# Autodesk Inventor assembly: Редуктор
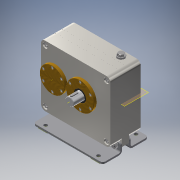
[picture p0: Inventor's stored thumbnail of the model, 180x180]
Saved by Autodesk Inventor 2016 (Build 200138000, 138)
## iProperties
Created: 2021-04-28
Part Number: Редуктор
Material: Типовые
Document SubType Name: Assembly
Designer: Лол
Mass: 4191.1 g
Surface Area: 9151.06 cm^2
Volume: 3369.82 cm^3
Density: 1.24372 g/cm^3
Author: Лол
## Documents named in this file (36)
- C:\Users\Лол\Documents\Inventor\course_work\Редуктор.iam
- C:\Users\Лол\Documents\Inventor\course_work\Корпус часть без резьбы.ipt
- C:\Users\Лол\Documents\Inventor\course_work\Подшипник\Подшипник-01.ipt
- C:\Users\Лол\Documents\Inventor\course_work\Подшипник.ipt
- C:\Users\Лол\Documents\Inventor\course_work\Подшипник\Подшипник-02.ipt
- C:\Users\Лол\Documents\Inventor\course_work\Быстроходный вал.ipt
- C:\Users\Лол\Documents\Inventor\course_work\Тихоходный вал.ipt
- C:\Users\Лол\Documents\Inventor\course_work\Кольцо A30 ГОСТ 13942-86.ipt
- C:\Users\Лол\Documents\Inventor\course_work\Кольцо A35 ГОСТ 13942-86.ipt
- C:\Users\Лол\Documents\Inventor\course_work\Тихоходное колесо.ipt
- C:\Users\Лол\Documents\Inventor\course_work\Корпус центральная часть.ipt
- C:\Users\Лол\Documents\Inventor\course_work\Корпус часть с резьбой.ipt
- C:\Users\Лол\Documents\Inventor\course_work\Гайка M30x1.5 6H ГОСТ 6393-73.ipt
- C:\Users\Лол\Documents\Inventor\course_work\Гайка M33x1.5 6H ГОСТ 6393-73.ipt
- C:\Users\Лол\Documents\Inventor\course_work\ISO 2340 - A - 6 x 40ISO.ipt
- C:\Users\Лол\Documents\Inventor\course_work\AS 1420 - 1973 - M10 x 75.ipt
- C:\Users\Лол\Documents\Inventor\course_work\Крышка маленькая_62.ipt
- C:\Users\Лол\Documents\Inventor\course_work\Крышка большая_72.ipt
- C:\Users\Лол\Documents\Inventor\course_work\AS 1420 - 1973 - M6 x 12.ipt
- C:\Users\Лол\Documents\Inventor\course_work\Крышка маленькая_под манж_01.ipt
- C:\Users\Лол\Documents\Inventor\course_work\Крышка большая_ПОД МАНЖЕТУ.ipt
- C:\Users\Лол\Documents\Inventor\course_work\Манжет 1-28x40x7 ГОСТ 8752-79.ipt
- C:\Users\Лол\Documents\Inventor\course_work\Манжет 1-30x42x7 ГОСТ 8752-79.ipt
- C:\Users\Лол\Documents\Inventor\course_work\ОПОРА_05.ipt
- C:\Users\Лол\Documents\Inventor\course_work\Шпонка 8x7x28 ГОСТ 23360-78.ipt
- C:\Users\Лол\Documents\Inventor\course_work\Болт 2 M10×50 ГОСТ 15591-70.ipt
- C:\Users\Лол\Documents\Inventor\course_work\Гайка M10-6H ГОСТ 5927-70.ipt
- C:\Users\Лол\Documents\Inventor\course_work\Шайба 2 10Л ГОСТ 6402-78.ipt
- C:\Users\Лол\Documents\Inventor\course_work\кол_062.ipt
- C:\Users\Лол\Documents\Inventor\course_work\кол_072.ipt
- C:\Users\Лол\Documents\Inventor\course_work\CSN 02 1915.21 - M 20 x 10.ipt
- C:\Users\Лол\Documents\Inventor\course_work\DIN 7603 - A22 x 27  (lt).ipt
- C:\Users\Лол\Documents\Inventor\course_work\платик под опору редуктора-01.ipt
- C:\Users\Лол\Documents\Inventor\course_work\Кольцо C6 ГОСТ 13942-86.ipt
- C:\Users\Лол\Documents\Inventor\course_work\ISO 2340 - A - 6 x 45ISO.ipt
- C:\Users\Лол\Documents\Inventor\course_work\сапун - M 20 x 10.ipt
## Components (82 placed, 33 different names)
1. Корпус часть без резьбы:1 — Заподлицо:1, Заподлицо:2, Заподлицо:3, Совмещение:1, Совмещение:2, Совмещение:3, Совмещение:4, Совмещение:14, Совмещение:28, Совмещение:33, Совмещение:34, Совмещение:35, Совмещение:36, Совмещение:37, Совмещение:38, Совмещение:39, Совмещение:40, Совмещение:43, Совмещение:44, Совмещение:61, Совмещение:62, Совмещение:82, Совмещение:83, Совмещение:84, Совмещение:191, Заподлицо:10, Совмещение:192, Заподлицо:11, Угол:1, Совмещение:215, Угол:14, Угол:15, Угол:16, Угол:17, Угол:18, Угол:19, Угол:20, Угол:21, Угол:22, Угол:23, Угол:27
2. Подшипник-01:1 — Совмещение:18, Совмещение:19, Совмещение:22, Совмещение:24, Совмещение:221
3. Подшипник-01:2 — Совмещение:1, Совмещение:2, Совмещение:5, Совмещение:13, Совмещение:222
4. Подшипник-02:3 — Совмещение:3, Совмещение:4, Совмещение:6, Совмещение:26, Совмещение:223
5. Подшипник-02:4 — Совмещение:16, Совмещение:17, Совмещение:, Совмещение:88, Совмещение:220
6. Быстроходный вал:1 — Совмещение:5, Совмещение:7, Совмещение:8, Совмещение:22, Совмещение:23, Совмещение:85, Совмещение:109, Совмещение:159, Совмещение:160, Угол:29
7. Тихоходный вал:1 — Совмещение:6, Совмещение:9, Совмещение:12, Совмещение:25, Совмещение:48, Совмещение:87, Совмещение:88, Совмещение:112, Совмещение:157, Совмещение:158
8. Кольцо A30 ГОСТ 13942-86:1 — Совмещение:7, Совмещение:8, Совмещение:13, Угол:27
9. Кольцо A35 ГОСТ 13942-86:1 — Совмещение:9, Совмещение:, Совмещение:48, Угол:26
10. Тихоходное колесо:2 — Совмещение:12, Совмещение:87, Угол:28
11. Корпус центральная часть:1 — Совмещение:14, Совмещение:15, Совмещение:30, Совмещение:32, Совмещение:114, Совмещение:115, Совмещение:116, Совмещение:117, Совмещение:118, Совмещение:119, Совмещение:161, Совмещение:168, Совмещение:173, Совмещение:174, Совмещение:209, Совмещение:210, Заподлицо:14, Совмещение:216, Угол:8, Угол:9, Угол:10, Угол:11, Угол:12, Угол:13, Совмещение:224, Угол:24, Угол:25
12. Корпус часть с резьбой:1 — Совмещение:15, Совмещение:16, Совмещение:17, Совмещение:18, Совмещение:19, Совмещение:49, Совмещение:56, Совмещение:57, Совмещение:65, Совмещение:79, Совмещение:80, Совмещение:81, Совмещение:187, Совмещение:188, Совмещение:189, Заподлицо:8, Совмещение:190, Заподлицо:9, Угол:2, Совмещение:195, Совмещение:199, Совмещение:200, Совмещение:217, Угол:7, Угол:26
13. Гайка M30x1.5 6H ГОСТ 6393-73:1 — Совмещение:23, Совмещение:24, Совмещение:225
14. Гайка M33x1.5 6H ГОСТ 6393-73:1 — Совмещение:25, Совмещение:26, Совмещение:226
15. ISO 2340 - A - 6 x 45ISO:1 — Совмещение:28, Совмещение:30, Совмещение:32
16. AS 1420 - 1973 - M10 x 75:1 — Совмещение:33, Совмещение:34, Совмещение:224, Угол:20
17. AS 1420 - 1973 - M10 x 75:2 — Совмещение:35, Совмещение:36, Угол:18
18. AS 1420 - 1973 - M10 x 75:3 — Совмещение:37, Совмещение:38, Угол:19
19. AS 1420 - 1973 - M10 x 75:4 — Совмещение:39, Совмещение:40, Угол:21
20. Крышка маленькая_62:1 — Совмещение:43, Совмещение:44, Совмещение:61, Совмещение:63, Совмещение:64
21. Крышка большая_72:2 — Совмещение:49, Совмещение:56, Совмещение:57, Совмещение:60, Совмещение:66
22. Крышка маленькая_под манж_01:1 — Совмещение:79, Совмещение:80, Совмещение:81, Заподлицо:6, Совмещение:107, Совмещение:108
23. Крышка большая_ПОД МАНЖЕТУ:1 — Совмещение:82, Совмещение:83, Совмещение:84, Заподлицо:7, Совмещение:86, Совмещение:110, Совмещение:111
24. Манжет 1-28x40x7 ГОСТ 8752-79:2 — Совмещение:85, Заподлицо:6
25. Манжет 1-30x42x7 ГОСТ 8752-79:1 — Заподлицо:7, Совмещение:86
26. ОПОРА_05:1 — Совмещение:114, Совмещение:115, Совмещение:116, Совмещение:162, Совмещение:167, Совмещение:175, Совмещение:176, Совмещение:205, Совмещение:206, Совмещение:207, Угол:5, Угол:6, Совмещение:208
27. ОПОРА_05:2 — Совмещение:117, Совмещение:118, Совмещение:119, Совмещение:164, Совмещение:170, Совмещение:177, Совмещение:178, Совмещение:201, Совмещение:202, Угол:3, Совмещение:203, Совмещение:204, Угол:4
28. Шпонка 8x7x28 ГОСТ 23360-78:1 — Совмещение:157, Совмещение:158, Угол:1
29. Шпонка 8x7x28 ГОСТ 23360-78:2 — Совмещение:159, Совмещение:160, Угол:2
30. Болт 2 M10×50 ГОСТ 15591-70:1 — Совмещение:173, Совмещение:175, Совмещение:179, Совмещение:183, Угол:12
31. Болт 2 M10×50 ГОСТ 15591-70:2 — Совмещение:167, Совмещение:168, Совмещение:169, Совмещение:172, Угол:11
32. Болт 2 M10×50 ГОСТ 15591-70:3 — Совмещение:174, Совмещение:176, Совмещение:180, Совмещение:184, Угол:13
33. Болт 2 M10×50 ГОСТ 15591-70:4 — Совмещение:161, Совмещение:162, Совмещение:163, Совмещение:165, Угол:10
34. Гайка M10-6H ГОСТ 5927-70:1 — Совмещение:165, Совмещение:166, Угол:17
35. Гайка M10-6H ГОСТ 5927-70:2 — Совмещение:184, Совмещение:185, Угол:14
36. Гайка M10-6H ГОСТ 5927-70:3 — Совмещение:183, Совмещение:186, Угол:15
37. Гайка M10-6H ГОСТ 5927-70:4 — Совмещение:171, Совмещение:172, Угол:16
38. Шайба 2 10Л ГОСТ 6402-78:1 — Совмещение:177, Совмещение:179, Совмещение:186
39. Шайба 2 10Л ГОСТ 6402-78:2 — Совмещение:178, Совмещение:180, Совмещение:185
40. Шайба 2 10Л ГОСТ 6402-78:3 — Совмещение:169, Совмещение:170, Совмещение:171
41. Шайба 2 10Л ГОСТ 6402-78:4 — Совмещение:163, Совмещение:164, Совмещение:166
42. кол_062:1 — Совмещение:187, Совмещение:188, Совмещение:189, Заподлицо:8
43. кол_062:2 — Совмещение:191, Заподлицо:10
44. кол_072:1 — Совмещение:192, Заподлицо:11
45. кол_072:2 — Совмещение:190, Заподлицо:9
46. CSN 02 1915.21 (мелкая резьба) M 20 x 10:1 — Совмещение:193, Совмещение:194, Совмещение:195, Угол:9
47. DIN 7603 A A22 x 27  (lt):1 — Совмещение:193, Совмещение:194, Совмещение:200
48. DIN 7603 A A22 x 27  (lt):2 — Совмещение:199, Совмещение:218
49. платик под опору редуктора-01:1 — Совмещение:201, Совмещение:202, Угол:3
50. платик под опору редуктора-01:2 — Совмещение:203, Совмещение:204, Угол:4
51. платик под опору редуктора-01:3 — Совмещение:206, Угол:6, Совмещение:208
52. платик под опору редуктора-01:4 — Совмещение:205, Совмещение:207, Угол:5
53. ISO 2340 - A - 6 x 40ISO:3 — Совмещение:209, Совмещение:211, Совмещение:213
54. ISO 2340 - A - 6 x 40ISO:4 — Совмещение:210, Совмещение:212, Совмещение:214
55. Кольцо C6 ГОСТ 13942-86:1 — Совмещение:211, Совмещение:213
56. Кольцо C6 ГОСТ 13942-86:2 — Совмещение:212, Совмещение:214, Совмещение:216
57. ISO 2340 - A - 6 x 45ISO:15 — Совмещение:215, Заподлицо:14
58. CSN 02 1915.21 (мелкая резьба) M 20 x 10:2 — Совмещение:217, Совмещение:218, Угол:7
59. AS 1420 - 1973 - M6 x 12:1 — Совмещение:62, Совмещение:63, Угол:22
60. AS 1420 - 1973 - M6 x 12:2
61. AS 1420 - 1973 - M6 x 12:3
62. AS 1420 - 1973 - M6 x 12:4
63. AS 1420 - 1973 - M6 x 12:5
64. AS 1420 - 1973 - M6 x 12:6
65. AS 1420 - 1973 - M6 x 12:8 — Совмещение:65, Совмещение:66, Угол:25
66. AS 1420 - 1973 - M6 x 12:9
67. AS 1420 - 1973 - M6 x 12:10
68. AS 1420 - 1973 - M6 x 12:11
69. AS 1420 - 1973 - M6 x 12:12
70. AS 1420 - 1973 - M6 x 12:13
71. AS 1420 - 1973 - M6 x 12:15 — Совмещение:107, Совмещение:108
72. AS 1420 - 1973 - M6 x 12:16
73. AS 1420 - 1973 - M6 x 12:17
74. AS 1420 - 1973 - M6 x 12:18 — Угол:24
75. AS 1420 - 1973 - M6 x 12:19
76. AS 1420 - 1973 - M6 x 12:20
77. AS 1420 - 1973 - M6 x 12:14 — Совмещение:110, Совмещение:111
78. AS 1420 - 1973 - M6 x 12:21
79. AS 1420 - 1973 - M6 x 12:22
80. AS 1420 - 1973 - M6 x 12:23 — Угол:23
81. AS 1420 - 1973 - M6 x 12:24
82. AS 1420 - 1973 - M6 x 12:25
## Component patterns: (6 elements, first: AS 1420 - 1973 - M6 x 12:1), (6 elements, first: AS 1420 - 1973 - M6 x 12:8), (6 elements, first: AS 1420 - 1973 - M6 x 12:15), (6 elements, first: AS 1420 - 1973 - M6 x 12:14)
## Relationships (173: Mate 134, Angle 29, Flush 10)
- Заподлицо:1 [Flush]: Корпус часть без резьбы:1
- Заподлицо:2 [Flush] (-37.142 mm): Корпус часть без резьбы:1
- Заподлицо:3 [Flush] (-27.571 mm): Корпус часть без резьбы:1
- Совмещение:1 [Mate]: Корпус часть без резьбы:1 ↔ Подшипник-01:2
- Совмещение:2 [Mate]: Корпус часть без резьбы:1 ↔ Подшипник-01:2
- Совмещение:3 [Mate]: Корпус часть без резьбы:1 ↔ Подшипник-02:3
- Совмещение:4 [Mate]: Корпус часть без резьбы:1 ↔ Подшипник-02:3
- Совмещение:5 [Mate]: Подшипник-01:2 ↔ Быстроходный вал:1
- Совмещение:6 [Mate]: Подшипник-02:3 ↔ Тихоходный вал:1
- Совмещение:7 [Mate]: Быстроходный вал:1 ↔ Кольцо A30 ГОСТ 13942-86:1
- Совмещение:8 [Mate]: Быстроходный вал:1 ↔ Кольцо A30 ГОСТ 13942-86:1
- Совмещение:9 [Mate]: Тихоходный вал:1 ↔ Кольцо A35 ГОСТ 13942-86:1
- Совмещение:12 [Mate]: Тихоходный вал:1 ↔ Тихоходное колесо:2
- Совмещение:13 [Mate]: Подшипник-01:2 ↔ Кольцо A30 ГОСТ 13942-86:1
- Совмещение:14 [Mate]: Корпус часть без резьбы:1 ↔ Корпус центральная часть:1
- Совмещение:15 [Mate]: Корпус центральная часть:1 ↔ Корпус часть с резьбой:1
- Совмещение:16 [Mate]: Подшипник-02:4 ↔ Корпус часть с резьбой:1
- Совмещение:17 [Mate]: Подшипник-02:4 ↔ Корпус часть с резьбой:1
- Совмещение:18 [Mate]: Подшипник-01:1 ↔ Корпус часть с резьбой:1
- Совмещение:19 [Mate]: Подшипник-01:1 ↔ Корпус часть с резьбой:1
- Совмещение: [Mate]: Подшипник-02:4 ↔ Кольцо A35 ГОСТ 13942-86:1
- Совмещение:22 [Mate]: Подшипник-01:1 ↔ Быстроходный вал:1
- Совмещение:23 [Mate]: Быстроходный вал:1 ↔ Гайка M30x1.5 6H ГОСТ 6393-73:1
- Совмещение:24 [Mate]: Подшипник-01:1 ↔ Гайка M30x1.5 6H ГОСТ 6393-73:1
- Совмещение:25 [Mate]: Тихоходный вал:1 ↔ Гайка M33x1.5 6H ГОСТ 6393-73:1
- Совмещение:26 [Mate]: Подшипник-02:3 ↔ Гайка M33x1.5 6H ГОСТ 6393-73:1
- Совмещение:28 [Mate]: Корпус часть без резьбы:1 ↔ ISO 2340 - A - 6 x 45ISO:1
- Совмещение:30 [Mate]: Корпус центральная часть:1 ↔ ISO 2340 - A - 6 x 45ISO:1
- Совмещение:32 [Mate] (10 mm): Корпус центральная часть:1 ↔ ISO 2340 - A - 6 x 45ISO:1
- Совмещение:33 [Mate]: Корпус часть без резьбы:1 ↔ AS 1420 - 1973 - M10 x 75:1
- Совмещение:34 [Mate]: Корпус часть без резьбы:1 ↔ AS 1420 - 1973 - M10 x 75:1
- Совмещение:35 [Mate]: Корпус часть без резьбы:1 ↔ AS 1420 - 1973 - M10 x 75:2
- Совмещение:36 [Mate]: Корпус часть без резьбы:1 ↔ AS 1420 - 1973 - M10 x 75:2
- Совмещение:37 [Mate]: Корпус часть без резьбы:1 ↔ AS 1420 - 1973 - M10 x 75:3
- Совмещение:38 [Mate]: Корпус часть без резьбы:1 ↔ AS 1420 - 1973 - M10 x 75:3
- Совмещение:39 [Mate]: Корпус часть без резьбы:1 ↔ AS 1420 - 1973 - M10 x 75:4
- Совмещение:40 [Mate]: Корпус часть без резьбы:1 ↔ AS 1420 - 1973 - M10 x 75:4
- Совмещение:43 [Mate]: Корпус часть без резьбы:1 ↔ Крышка маленькая_62:1
- Совмещение:44 [Mate]: Корпус часть без резьбы:1 ↔ Крышка маленькая_62:1
- Совмещение:48 [Mate]: Тихоходный вал:1 ↔ Кольцо A35 ГОСТ 13942-86:1
- Совмещение:49 [Mate]: Корпус часть с резьбой:1 ↔ Крышка большая_72:2
- Совмещение:56 [Mate]: Корпус часть с резьбой:1 ↔ Крышка большая_72:2
- Совмещение:57 [Mate]: Корпус часть с резьбой:1 ↔ Крышка большая_72:2
- Совмещение:60 [Mate]: Крышка большая_72:2
- Совмещение:61 [Mate]: Корпус часть без резьбы:1 ↔ Крышка маленькая_62:1
- Совмещение:62 [Mate]: Корпус часть без резьбы:1 ↔ AS 1420 - 1973 - M6 x 12:1
- Совмещение:63 [Mate]: Крышка маленькая_62:1 ↔ AS 1420 - 1973 - M6 x 12:1
- Совмещение:64 [Mate]: Крышка маленькая_62:1
- Совмещение:65 [Mate]: Корпус часть с резьбой:1 ↔ AS 1420 - 1973 - M6 x 12:8
- Совмещение:66 [Mate]: Крышка большая_72:2 ↔ AS 1420 - 1973 - M6 x 12:8
- Совмещение:79 [Mate]: Корпус часть с резьбой:1 ↔ Крышка маленькая_под манж_01:1
- Совмещение:80 [Mate]: Корпус часть с резьбой:1 ↔ Крышка маленькая_под манж_01:1
- Совмещение:81 [Mate]: Корпус часть с резьбой:1 ↔ Крышка маленькая_под манж_01:1
- Совмещение:82 [Mate]: Корпус часть без резьбы:1 ↔ Крышка большая_ПОД МАНЖЕТУ:1
- Совмещение:83 [Mate]: Корпус часть без резьбы:1 ↔ Крышка большая_ПОД МАНЖЕТУ:1
- Совмещение:84 [Mate]: Корпус часть без резьбы:1 ↔ Крышка большая_ПОД МАНЖЕТУ:1
- Совмещение:85 [Mate]: Быстроходный вал:1 ↔ Манжет 1-28x40x7 ГОСТ 8752-79:2
- Заподлицо:6 [Flush]: Крышка маленькая_под манж_01:1 ↔ Манжет 1-28x40x7 ГОСТ 8752-79:2
- Заподлицо:7 [Flush]: Крышка большая_ПОД МАНЖЕТУ:1 ↔ Манжет 1-30x42x7 ГОСТ 8752-79:1
- Совмещение:86 [Mate]: Крышка большая_ПОД МАНЖЕТУ:1 ↔ Манжет 1-30x42x7 ГОСТ 8752-79:1
- Совмещение:87 [Mate]: Тихоходный вал:1 ↔ Тихоходное колесо:2
- Совмещение:88 [Mate]: Подшипник-02:4 ↔ Тихоходный вал:1
- Совмещение:107 [Mate]: Крышка маленькая_под манж_01:1 ↔ AS 1420 - 1973 - M6 x 12:15
- Совмещение:108 [Mate]: Крышка маленькая_под манж_01:1 ↔ AS 1420 - 1973 - M6 x 12:15
- Совмещение:109 [Mate]: Быстроходный вал:1
- Совмещение:110 [Mate]: Крышка большая_ПОД МАНЖЕТУ:1 ↔ AS 1420 - 1973 - M6 x 12:14
- Совмещение:111 [Mate]: Крышка большая_ПОД МАНЖЕТУ:1 ↔ AS 1420 - 1973 - M6 x 12:14
- Совмещение:112 [Mate]: Тихоходный вал:1
- Совмещение:114 [Mate]: Корпус центральная часть:1 ↔ ОПОРА_05:1
- Совмещение:115 [Mate]: Корпус центральная часть:1 ↔ ОПОРА_05:1
- Совмещение:116 [Mate]: Корпус центральная часть:1 ↔ ОПОРА_05:1
- Совмещение:117 [Mate]: Корпус центральная часть:1 ↔ ОПОРА_05:2
- Совмещение:118 [Mate]: Корпус центральная часть:1 ↔ ОПОРА_05:2
- Совмещение:119 [Mate]: Корпус центральная часть:1 ↔ ОПОРА_05:2
- Совмещение:157 [Mate]: Тихоходный вал:1 ↔ Шпонка 8x7x28 ГОСТ 23360-78:1
- Совмещение:158 [Mate]: Тихоходный вал:1 ↔ Шпонка 8x7x28 ГОСТ 23360-78:1
- Совмещение:159 [Mate]: Быстроходный вал:1 ↔ Шпонка 8x7x28 ГОСТ 23360-78:2
- Совмещение:160 [Mate]: Быстроходный вал:1 ↔ Шпонка 8x7x28 ГОСТ 23360-78:2
- Совмещение:161 [Mate]: Корпус центральная часть:1 ↔ Болт 2 M10×50 ГОСТ 15591-70:4
- Совмещение:162 [Mate]: ОПОРА_05:1 ↔ Болт 2 M10×50 ГОСТ 15591-70:4
- Совмещение:163 [Mate]: Болт 2 M10×50 ГОСТ 15591-70:4 ↔ Шайба 2 10Л ГОСТ 6402-78:4
- Совмещение:164 [Mate]: ОПОРА_05:2 ↔ Шайба 2 10Л ГОСТ 6402-78:4
- Совмещение:165 [Mate]: Болт 2 M10×50 ГОСТ 15591-70:4 ↔ Гайка M10-6H ГОСТ 5927-70:1
- Совмещение:166 [Mate]: Гайка M10-6H ГОСТ 5927-70:1 ↔ Шайба 2 10Л ГОСТ 6402-78:4
- Совмещение:167 [Mate]: ОПОРА_05:1 ↔ Болт 2 M10×50 ГОСТ 15591-70:2
- Совмещение:168 [Mate]: Корпус центральная часть:1 ↔ Болт 2 M10×50 ГОСТ 15591-70:2
- Совмещение:169 [Mate]: Болт 2 M10×50 ГОСТ 15591-70:2 ↔ Шайба 2 10Л ГОСТ 6402-78:3
- Совмещение:170 [Mate]: ОПОРА_05:2 ↔ Шайба 2 10Л ГОСТ 6402-78:3
- Совмещение:171 [Mate]: Гайка M10-6H ГОСТ 5927-70:4 ↔ Шайба 2 10Л ГОСТ 6402-78:3
- Совмещение:172 [Mate]: Болт 2 M10×50 ГОСТ 15591-70:2 ↔ Гайка M10-6H ГОСТ 5927-70:4
- Совмещение:173 [Mate]: Корпус центральная часть:1 ↔ Болт 2 M10×50 ГОСТ 15591-70:1
- Совмещение:174 [Mate]: Корпус центральная часть:1 ↔ Болт 2 M10×50 ГОСТ 15591-70:3
- Совмещение:175 [Mate]: ОПОРА_05:1 ↔ Болт 2 M10×50 ГОСТ 15591-70:1
- Совмещение:176 [Mate]: ОПОРА_05:1 ↔ Болт 2 M10×50 ГОСТ 15591-70:3
- Совмещение:177 [Mate]: ОПОРА_05:2 ↔ Шайба 2 10Л ГОСТ 6402-78:1
- Совмещение:178 [Mate]: ОПОРА_05:2 ↔ Шайба 2 10Л ГОСТ 6402-78:2
- Совмещение:179 [Mate]: Болт 2 M10×50 ГОСТ 15591-70:1 ↔ Шайба 2 10Л ГОСТ 6402-78:1
- Совмещение:180 [Mate]: Болт 2 M10×50 ГОСТ 15591-70:3 ↔ Шайба 2 10Л ГОСТ 6402-78:2
- Совмещение:183 [Mate]: Болт 2 M10×50 ГОСТ 15591-70:1 ↔ Гайка M10-6H ГОСТ 5927-70:3
- Совмещение:184 [Mate]: Болт 2 M10×50 ГОСТ 15591-70:3 ↔ Гайка M10-6H ГОСТ 5927-70:2
- Совмещение:185 [Mate]: Гайка M10-6H ГОСТ 5927-70:2 ↔ Шайба 2 10Л ГОСТ 6402-78:2
- Совмещение:186 [Mate]: Гайка M10-6H ГОСТ 5927-70:3 ↔ Шайба 2 10Л ГОСТ 6402-78:1
- Совмещение:187 [Mate]: Корпус часть с резьбой:1 ↔ кол_062:1
- Совмещение:188 [Mate]: Корпус часть с резьбой:1 ↔ кол_062:1
- Совмещение:189 [Mate]: Корпус часть с резьбой:1 ↔ кол_062:1
- Заподлицо:8 [Flush]: Корпус часть с резьбой:1 ↔ кол_062:1
- Совмещение:190 [Mate]: Корпус часть с резьбой:1 ↔ кол_072:2
- Заподлицо:9 [Flush]: Корпус часть с резьбой:1 ↔ кол_072:2
- Совмещение:191 [Mate]: Корпус часть без резьбы:1 ↔ кол_062:2
- Заподлицо:10 [Flush]: Корпус часть без резьбы:1 ↔ кол_062:2
- Совмещение:192 [Mate]: Корпус часть без резьбы:1 ↔ кол_072:1
- Заподлицо:11 [Flush]: Корпус часть без резьбы:1 ↔ кол_072:1
- Угол:1 [Angle] (0 deg): Корпус часть без резьбы:1 ↔ Шпонка 8x7x28 ГОСТ 23360-78:1
- Угол:2 [Angle] (0 deg): Корпус часть с резьбой:1 ↔ Шпонка 8x7x28 ГОСТ 23360-78:2
- Совмещение:193 [Mate]: CSN 02 1915.21 (мелкая резьба) M 20 x 10:1 ↔ DIN 7603 A A22 x 27  (lt):1
- Совмещение:194 [Mate]: CSN 02 1915.21 (мелкая резьба) M 20 x 10:1 ↔ DIN 7603 A A22 x 27  (lt):1
- Совмещение:195 [Mate]: Корпус часть с резьбой:1 ↔ CSN 02 1915.21 (мелкая резьба) M 20 x 10:1
- Совмещение:199 [Mate]: Корпус часть с резьбой:1 ↔ DIN 7603 A A22 x 27  (lt):2
- Совмещение:200 [Mate]: Корпус часть с резьбой:1 ↔ DIN 7603 A A22 x 27  (lt):1
- Совмещение:201 [Mate]: ОПОРА_05:2 ↔ платик под опору редуктора-01:1
- Совмещение:202 [Mate]: ОПОРА_05:2 ↔ платик под опору редуктора-01:1
- Угол:3 [Angle] (0 deg): ОПОРА_05:2 ↔ платик под опору редуктора-01:1
- Совмещение:203 [Mate]: ОПОРА_05:2 ↔ платик под опору редуктора-01:2
- Совмещение:204 [Mate]: ОПОРА_05:2 ↔ платик под опору редуктора-01:2
- Угол:4 [Angle] (0 deg): ОПОРА_05:2 ↔ платик под опору редуктора-01:2
- Совмещение:205 [Mate]: ОПОРА_05:1 ↔ платик под опору редуктора-01:4
- Совмещение:206 [Mate]: ОПОРА_05:1 ↔ платик под опору редуктора-01:3
- Совмещение:207 [Mate]: ОПОРА_05:1 ↔ платик под опору редуктора-01:4
- Угол:5 [Angle] (0 deg): ОПОРА_05:1 ↔ платик под опору редуктора-01:4
- Угол:6 [Angle] (0 deg): ОПОРА_05:1 ↔ платик под опору редуктора-01:3
- Совмещение:208 [Mate]: ОПОРА_05:1 ↔ платик под опору редуктора-01:3
- Совмещение:209 [Mate]: Корпус центральная часть:1 ↔ ISO 2340 - A - 6 x 40ISO:3
- Совмещение:210 [Mate]: Корпус центральная часть:1 ↔ ISO 2340 - A - 6 x 40ISO:4
- Совмещение:211 [Mate]: ISO 2340 - A - 6 x 40ISO:3 ↔ Кольцо C6 ГОСТ 13942-86:1
- Совмещение:212 [Mate]: ISO 2340 - A - 6 x 40ISO:4 ↔ Кольцо C6 ГОСТ 13942-86:2
- Совмещение:213 [Mate]: ISO 2340 - A - 6 x 40ISO:3 ↔ Кольцо C6 ГОСТ 13942-86:1
- Совмещение:214 [Mate]: ISO 2340 - A - 6 x 40ISO:4 ↔ Кольцо C6 ГОСТ 13942-86:2
- Совмещение:215 [Mate]: Корпус часть без резьбы:1 ↔ ISO 2340 - A - 6 x 45ISO:15
- Заподлицо:14 [Flush] (-10 mm): Корпус центральная часть:1 ↔ ISO 2340 - A - 6 x 45ISO:15
- Совмещение:216 [Mate]: Корпус центральная часть:1 ↔ Кольцо C6 ГОСТ 13942-86:2
- Совмещение:217 [Mate]: Корпус часть с резьбой:1 ↔ CSN 02 1915.21 (мелкая резьба) M 20 x 10:2
- Совмещение:218 [Mate]: DIN 7603 A A22 x 27  (lt):2 ↔ CSN 02 1915.21 (мелкая резьба) M 20 x 10:2
- Угол:7 [Angle] (0 deg): Корпус часть с резьбой:1 ↔ CSN 02 1915.21 (мелкая резьба) M 20 x 10:2
- Совмещение:219 [Mate]
- Угол:8 [Angle] (90 deg): Корпус центральная часть:1
- Совмещение:220 [Mate]: Подшипник-02:4
- Совмещение:221 [Mate]: Подшипник-01:1
- Совмещение:222 [Mate]: Подшипник-01:2
- Совмещение:223 [Mate]: Подшипник-02:3
- Угол:9 [Angle] (0 deg): Корпус центральная часть:1 ↔ CSN 02 1915.21 (мелкая резьба) M 20 x 10:1
- Угол:10 [Angle] (0 deg): Корпус центральная часть:1 ↔ Болт 2 M10×50 ГОСТ 15591-70:4
- Угол:11 [Angle] (0 deg): Корпус центральная часть:1 ↔ Болт 2 M10×50 ГОСТ 15591-70:2
- Угол:12 [Angle] (0 deg): Корпус центральная часть:1 ↔ Болт 2 M10×50 ГОСТ 15591-70:1
- Угол:13 [Angle] (0 deg): Корпус центральная часть:1 ↔ Болт 2 M10×50 ГОСТ 15591-70:3
- Угол:14 [Angle] (0 deg): Корпус часть без резьбы:1 ↔ Гайка M10-6H ГОСТ 5927-70:2
- Угол:15 [Angle] (0 deg): Корпус часть без резьбы:1 ↔ Гайка M10-6H ГОСТ 5927-70:3
- Совмещение:224 [Mate]: Корпус центральная часть:1 ↔ AS 1420 - 1973 - M10 x 75:1
- Угол:16 [Angle] (0 deg): Корпус часть без резьбы:1 ↔ Гайка M10-6H ГОСТ 5927-70:4
- Угол:17 [Angle] (0 deg): Корпус часть без резьбы:1 ↔ Гайка M10-6H ГОСТ 5927-70:1
- Угол:18 [Angle] (0 deg): Корпус часть без резьбы:1 ↔ AS 1420 - 1973 - M10 x 75:2
- Угол:19 [Angle] (0 deg): Корпус часть без резьбы:1 ↔ AS 1420 - 1973 - M10 x 75:3
- Угол:20 [Angle] (0 deg): Корпус часть без резьбы:1 ↔ AS 1420 - 1973 - M10 x 75:1
- Угол:21 [Angle] (0 deg): Корпус часть без резьбы:1 ↔ AS 1420 - 1973 - M10 x 75:4
- Угол:22 [Angle] (180 deg): Корпус часть без резьбы:1 ↔ AS 1420 - 1973 - M6 x 12:1
- Угол:23 [Angle] (180 deg): Корпус часть без резьбы:1 ↔ AS 1420 - 1973 - M6 x 12:23
- Угол:24 [Angle] (180 deg): Корпус центральная часть:1 ↔ AS 1420 - 1973 - M6 x 12:18
- Угол:25 [Angle] (180 deg): Корпус центральная часть:1 ↔ AS 1420 - 1973 - M6 x 12:8
- Совмещение:225 [Mate]: Гайка M30x1.5 6H ГОСТ 6393-73:1
- Совмещение:226 [Mate]: Гайка M33x1.5 6H ГОСТ 6393-73:1
- Угол:26 [Angle] (0 deg): Кольцо A35 ГОСТ 13942-86:1 ↔ Корпус часть с резьбой:1
- Угол:27 [Angle] (0 deg): Корпус часть без резьбы:1 ↔ Кольцо A30 ГОСТ 13942-86:1
- Угол:28 [Angle] (0 deg): Тихоходное колесо:2
- Угол:29 [Angle] (0 deg): Быстроходный вал:1
